# Autodesk Inventor assembly: chamber_assembly
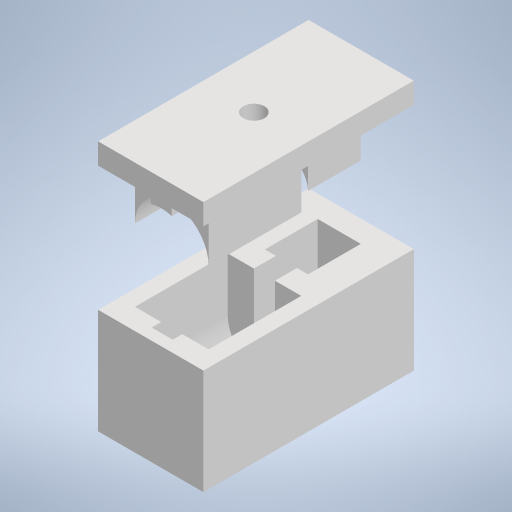
[picture p0: Inventor's stored thumbnail of the model, 512x512]
Saved by Autodesk Inventor 2023 (Build 270158000, 158)
## iProperties
Created: 2023-03-20
Part Number: chamber_assembly
Document SubType Name: Assembly
Designer: caleb
Author: caleb
## Documents named in this file (3)
- C:\Users\caleb\Documents\Inventor\SPICE\chamber_assembly.iam
- C:\Users\caleb\Documents\Inventor\SPICE\dcmotor_housing.ipt
- C:\Users\caleb\Documents\Inventor\SPICE\dcmotor_housing_lid.ipt
## Components (2 placed, 2 different names)
1. dcmotor_housing:1 — Flush:1, Flush:2
2. dcmotor_housing_lid:1 — Flush:1, Flush:2
## Relationships (2: Flush 2)
- Flush:1: dcmotor_housing:1 ↔ dcmotor_housing_lid:1
- Flush:2: dcmotor_housing:1 ↔ dcmotor_housing_lid:1
